# Autodesk Inventor assembly: Assembly1
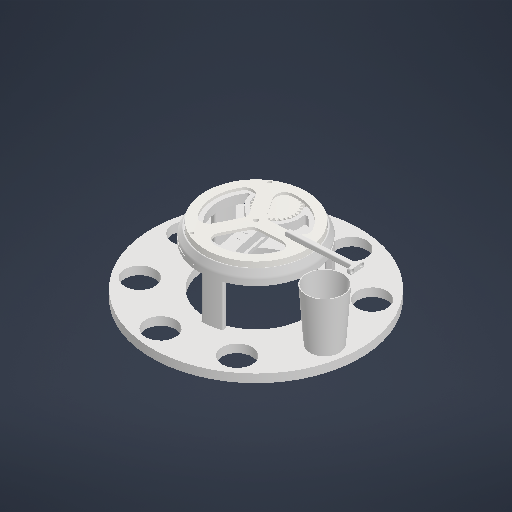
[picture p0: Inventor's stored thumbnail of the model, 512x512]
Saved by Autodesk Inventor 2026.2 (Build 302298000, 298)
## iProperties
Created: 2026-01-26
Part Number: Assembly1
Document SubType Name: Assembly
Designer: Cobble
Author: Cobble
## Documents named in this file (10)
- D:\CAD\Shot Filler V3\Assembly1.iam
- D:\CAD\Shot Filler V3\Gear Holder 1.ipt
- D:\CAD\Shot Filler V3\Gear Holder 2.ipt
- D:\CAD\Shot Filler V3\Assembly1\Design Accelerator\Spur Gear12.ipt
- D:\CAD\Shot Filler V3\Assembly1\Design Accelerator\Spur Gear22.ipt
- D:\CAD\Shot Filler V3\Part1.ipt
- D:\CAD\Shot Filler V3\Stand.ipt
- D:\CAD\Shotglass_Ref.ipt
- D:\CAD\Shot Filler V3\Cover.ipt
- D:\CAD\Shot Filler V3\Arm.ipt
## Components (9 placed, 9 different names)
1. Gear Holder 1:1 — Mate:3, Mate:4, Insert:4, Insert:5
2. Gear Holder 2:1 — Mate:3, Insert:3, Mate:4, Insert:4, Insert:6, Rotation:2
3. Spur Gear1:1 — Rotation:1, Insert:3
4. Spur Gear2:1 — Rotation:1, Insert:5, Insert:8, Insert:9
5. Part1:1 — Mate:5, Mate:6, Flush:1, Insert:7
6. Stand:1 — Mate:5, Mate:6, Insert:6, Flush:1, Rotation:2
7. Shotglass_Ref:1 — Insert:7
8. Cover:1 — Insert:8, Insert:9, Mate:7, Mate:8
9. Arm:1 — Mate:7, Mate:8
## Relationships (16: Insert 7, Mate 6, RelateRotation 2, Flush 1)
- Mate:3: Gear Holder 1:1 ↔ Gear Holder 2:1
- Rotation:1 [RelateRotation] (2.4839 ul): Spur Gear1:1 ↔ Spur Gear2:1
- Insert:3: Gear Holder 2:1 ↔ Spur Gear1:1
- Mate:4: Gear Holder 1:1 ↔ Gear Holder 2:1
- Insert:4: Gear Holder 1:1 ↔ Gear Holder 2:1
- Insert:5: Gear Holder 1:1 ↔ Spur Gear2:1
- Mate:5: Part1:1 ↔ Stand:1
- Mate:6: Part1:1 ↔ Stand:1
- Insert:6: Gear Holder 2:1 ↔ Stand:1
- Flush:1: Part1:1 ↔ Stand:1
- Rotation:2 [RelateRotation] (1 ul): Gear Holder 2:1 ↔ Stand:1
- Insert:7: Part1:1 ↔ Shotglass_Ref:1
- Insert:8: Spur Gear2:1 ↔ Cover:1
- Insert:9: Spur Gear2:1 ↔ Cover:1
- Mate:7: Cover:1 ↔ Arm:1
- Mate:8: Cover:1 ↔ Arm:1
